# Autodesk Inventor assembly: modularRICH
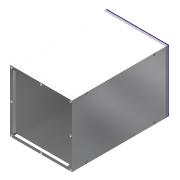
[picture p0: Inventor's stored thumbnail of the model, 180x180]
Saved by Autodesk Inventor 2018 (Build 220112000, 112)
## iProperties
Created: 2015-10-13
Part Number: modularRICH
Document SubType Name: Assembly
Designer: Sawaiz
Author: Sawaiz
## Documents named in this file (9)
- C:\Users\sawaiz\OneDrive\projects\modularRICH\modularRICH.iam
- C:\Users\sawaiz\OneDrive\projects\modularRICH\frame\frame.iam
- C:\Users\sawaiz\OneDrive\projects\modularRICH\fresnelLens.ipt
- C:\Users\sawaiz\OneDrive\projects\modularRICH\mirror\mirrorHolder.iam
- C:\Users\sawaiz\OneDrive\projects\modularRICH\aerogel.ipt
- C:\Users\sawaiz\OneDrive\projects\modularRICH\aerogelHolder.ipt
- C:\Users\sawaiz\OneDrive\projects\modularRICH\dependency\modularRICHBackplane\cad\detectorArray.iam
- C:\Users\sawaiz\OneDrive\projects\modularRICH\hardware\4-40x0.5in-pan.ipt
- C:\Users\sawaiz\OneDrive\projects\modularRICH\modularRICH.xlsx
## Components (10 placed, 7 different names)
1. frame:1 [sub-assembly] — Angle:1, Mate:3, Mate:7, Mate:8, Mate:10, Flush:3, Flush:4, Mate:18, Mate:19, Mate:21, Mate:22, Mate:23, Mate:24, Mate:25
2. mirrorHolder:1 [sub-assembly] — Mate:10, Mate:21, Mate:23
3. fresnelLens:1 — Mate:18, Mate:19, Mate:22
4. aerogel:1 — Mate:1, Mate:2, Flush:1
5. aerogelHolder:1 — Angle:1, Mate:1, Mate:2, Flush:1, Mate:3, Mate:7, Mate:8, Mate:25
6. detectorArray:1 [sub-assembly] — Flush:3, Flush:4, Mate:13, Mate:14, Mate:15, Mate:16, Mate:17, Mate:24
7. 4-40x0.5in-pan:1 — Mate:13, Flush:7
8. 4-40x0.5in-pan:2 — Mate:14, Flush:6
9. 4-40x0.5in-pan:3 — Mate:16, Flush:5, Flush:6, Flush:7, Mate:17
10. 4-40x0.5in-pan:4 — Mate:15, Flush:5
## Relationships (25: Mate 18, Flush 6, Angle 1)
- Angle:1 (0 deg): frame:1 ↔ aerogelHolder:1
- Mate:1: aerogel:1 ↔ aerogelHolder:1
- Mate:2: aerogel:1 ↔ aerogelHolder:1
- Flush:1: aerogel:1 ↔ aerogelHolder:1
- Mate:3: frame:1 ↔ aerogelHolder:1
- Mate:7: frame:1 ↔ aerogelHolder:1
- Mate:8: frame:1 ↔ aerogelHolder:1
- Mate:10 (0.1016 mm): frame:1 ↔ mirrorHolder:1
- Flush:3: frame:1 ↔ detectorArray:1
- Flush:4: frame:1 ↔ detectorArray:1
- Mate:13: detectorArray:1 ↔ 4-40x0.5in-pan:1
- Mate:14: detectorArray:1 ↔ 4-40x0.5in-pan:2
- Mate:15: detectorArray:1 ↔ 4-40x0.5in-pan:4
- Mate:16: detectorArray:1 ↔ 4-40x0.5in-pan:3
- Flush:5: 4-40x0.5in-pan:3 ↔ 4-40x0.5in-pan:4
- Flush:6: 4-40x0.5in-pan:2 ↔ 4-40x0.5in-pan:3
- Flush:7: 4-40x0.5in-pan:1 ↔ 4-40x0.5in-pan:3
- Mate:17: detectorArray:1 ↔ 4-40x0.5in-pan:3
- Mate:18 (0.0317 mm): frame:1 ↔ fresnelLens:1
- Mate:19 (0.0508 mm): frame:1 ↔ fresnelLens:1
- Mate:21 (0.1016 mm): frame:1 ↔ mirrorHolder:1
- Mate:22 (0.1016 mm): frame:1 ↔ fresnelLens:1
- Mate:23 (0.0508 mm): frame:1 ↔ mirrorHolder:1
- Mate:24: frame:1 ↔ detectorArray:1
- Mate:25: frame:1 ↔ aerogelHolder:1
## Named parameters: acrylicThickness = 6.35 mm, aerogelThickness = 30 mm, height = 127 mm, width = 127 mm, depth = 203.2 mm, mirrorAngle = 2.5 deg, detectorWidth = 52 mm, detectorHeight = 52 mm, mirrorThickness = 3.175 mm, fresnelThickness = 0.254 mm, grooveDensity = 125, focalLength = 152.4 mm, ior = 1.49, centerThickness = 1.27 mm, fresnelAngle = 90 deg, fresnelEffectiveDiameter = 152.4 mm, mirrorSuppourtWidth = 38.1 mm, backGrooveBit = 4.8006 mm, sensorHolderWidth = 88.9 mm, sensorHolderSesnorHeight = 53.975 mm, sensorHolderSensorWidth = 53.975 mm, sensorHolderHeight = 88.9 mm, sensorHolderSensorHeight = 53.975 mm, sensorHolderORingGroove = 3.175 mm, sensorHolderORing = 3.175 mm, sensorHolderFlushORingID = 304.8 mm, sensorHolderFlushORing = 3.175 mm, oRingWidth = 1.5875 mm, sensorHolderORingID = 203.2 mm, frontBackORingID = 419.1 mm, topBottomHorizontalMirrorGroove = 12.7 mm, backMirrorGroove = 6.35 mm, mirrorGroove = 19.05 mm, compressionPercent = 40, fresnelChamfer = 6.35 mm, mirrorGrooveFillet = 6.35 mm, mirrorGrooveDrill = 6.35 mm, mirrorGrooveMill = 3.175 mm, fresnelMirrorChamfer = 6.35 mm, detectorOpeningHeight = 76.2 mm, detectorOpeningWidth = 76.2 mm, sensorHolderDepth = 19.05 mm, aerogelHeight = 110 mm, aerogelWidth = 110 mm, frameAcrylicThickness = 9.525 mm, internalAcrylicThicnkess = 6.35 mm, internalAcrylicThickness = 6.35 mm, aerogelClearence = 3.175 mm, backplanePCBWidth = 76.2 mm, backplanePCBHeight = 76.2 mm, backplaneHoleOffsett = 6.35 mm, backplanePostionOffsett = 12.7 mm, moduleSlotClearence = 0.79375 mm, testMountWidth = 300 mm, testMountHeight = 300 mm, testMountLength = 500 mm, aerogelHolderDepth = 49.022 mm, plasticThickness = 6.35 mm, caseThickness = 6.35 mm, alignmentGrooveDepth = 1.5875 mm, alignmentGrooveClearance = 0.1016 mm, frontPanelThickness = 1.5875 mm, fresnelGrooveWidth = 1.778 mm
